# Autodesk Inventor assembly: Return_Spool_Mount
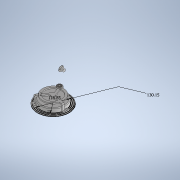
[picture p0: Inventor's stored thumbnail of the model, 180x180]
Saved by Autodesk Inventor 2022 (Build 260153070, 153G)
## iProperties
Created: 2022-03-05
Part Number: Return_Spool_Mount
Document SubType Name: Assembly
Designer: a laptop
Author: a laptop
## Documents named in this file (7)
- C:\Users\a laptop\Desktop\MDL_2021_Project\Return_Spool_Reel\Return_Spool_Mount.iam
- C:\Users\a laptop\Desktop\MDL_2021_Project\Return_Spool_Reel\Return_Spool_Mount.ipt
- C:\Users\a laptop\Desktop\MDL_2021_Project\Return_Spool_Reel\Screws\M8 Washer98689A116_General Purpose 18-8 Stainless Steel Washer.ipt
- C:\Users\a laptop\Desktop\MDL_2021_Project\Return_Spool_Reel\Return_Spool_Mount\Design Accelerator\Bearing2.iam
- C:\Users\a laptop\Desktop\MDL_2021_Project\Return_Spool_Reel\SRM-12-06A.ipt
- C:\Users\a laptop\Desktop\MDL_2021_Project\Return_Spool_Reel\Return_Spool.ipt
- C:\Users\a laptop\Desktop\MDL_2021_Project\Return_Spool_Reel\Bearing_Mount.ipt
## Components (6 placed, 6 different names)
1. Return_Spool_Mount:1 — Mate:19, Mate:20, Mate:21
2. Bearing:1 [sub-assembly] — Mate:15, Mate:16, Mate:23
3. SRM-12-06A:1 — Mate:11, Mate:18, Mate:19, Mate:20, Mate:21, Mate:22
4. Return_Spool:1 — Mate:16, Mate:17
5. Bearing_Mount:1 — Mate:11, Mate:13, Mate:14, Mate:17, Mate:18, Mate:22, Mate:23
6. M8 Washer98689A116_General Purpose 18-8 Stainless Steel Washer:1 — Mate:13, Mate:14, Mate:15
## Relationships (12: Mate 12)
- Mate:11: SRM-12-06A:1 ↔ Bearing_Mount:1
- Mate:13: Bearing_Mount:1 ↔ M8 Washer98689A116_General Purpose 18-8 Stainless Steel Washer:1
- Mate:14: Bearing_Mount:1 ↔ M8 Washer98689A116_General Purpose 18-8 Stainless Steel Washer:1
- Mate:15: Bearing:1 ↔ M8 Washer98689A116_General Purpose 18-8 Stainless Steel Washer:1
- Mate:16: Bearing:1 ↔ Return_Spool:1
- Mate:17: Return_Spool:1 ↔ Bearing_Mount:1
- Mate:18: SRM-12-06A:1 ↔ Bearing_Mount:1
- Mate:19: Return_Spool_Mount:1 ↔ SRM-12-06A:1
- Mate:20: Return_Spool_Mount:1 ↔ SRM-12-06A:1
- Mate:21: Return_Spool_Mount:1 ↔ SRM-12-06A:1
- Mate:22: SRM-12-06A:1 ↔ Bearing_Mount:1
- Mate:23: Bearing:1 ↔ Bearing_Mount:1
